# Autodesk Inventor assembly: Ribbon Cable Male Both Directions
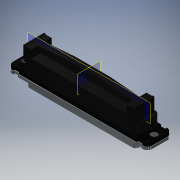
[picture p0: Inventor's stored thumbnail of the model, 180x180]
Saved by Autodesk Inventor 2019 (Build 230136000, 136)
## iProperties
Created: 2019-02-06
Part Number: Ribbon Cable Male Both Directions
Document SubType Name: Assembly
Designer: Serge
Author: Serge
## Documents named in this file (3)
- C:\Users\Serge\Desktop\Ribbon Cable\Ribbon Cable Male Both Directions.iam
- C:\Users\Serge\Desktop\Ribbon Cable\Dsub 37 Pin, 2 Row, Male.ipt
- C:\Users\Serge\Desktop\Ribbon Cable\Ribbon Mount Both Directions.ipt
## Components (2 placed, 2 different names)
1. Dsub 37 Pin, 2 Row, Male:1 — Mate:1, Flush:1, Flush:2
2. Ribbon Mount Both Directions:1 — Mate:1, Flush:1, Flush:2
## Relationships (3: Flush 2, Mate 1)
- Mate:1: Dsub 37 Pin, 2 Row, Male:1 ↔ Ribbon Mount Both Directions:1
- Flush:1 (7 mm): Dsub 37 Pin, 2 Row, Male:1 ↔ Ribbon Mount Both Directions:1
- Flush:2: Dsub 37 Pin, 2 Row, Male:1 ↔ Ribbon Mount Both Directions:1
